# Autodesk Inventor assembly: motor_GM1806-80T_skyProRO
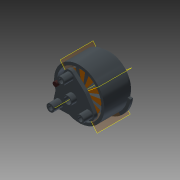
[picture p0: Inventor's stored thumbnail of the model, 180x180]
Saved by Autodesk Inventor 2015 SP1 (Build 190203100, 203)
## iProperties
Created: 2015-08-06
Part Number: motor_GM1806-80T_skyProRO
Document SubType Name: Assembly
Designer: Alexandre Cherpillod
Mass: 18 g
Surface Area: 55.0116 cm^2
Volume: 3.08775 cm^3
Author: Alexandre Cherpillod
## Documents named in this file (3)
- D:\_windows\_github_doc\MAVRIC\Mechanics\myCopter_CAD\Inventor\Gimbal_Brushless\motor_GM1806-80T_skyPro.iam
- D:\_windows\_github_doc\MAVRIC\Mechanics\myCopter_CAD\Inventor\Gimbal_Brushless\motor_GM1806-80T_Skypro_stator.ipt
- D:\_windows\_github_doc\MAVRIC\Mechanics\myCopter_CAD\Inventor\Gimbal_Brushless\motor_GM1806-80T_Skypro_rotor.ipt
## Components (2 placed, 2 different names)
1. motor_GM1806-80T_Skypro_stator:1 — Mate:1, Mate:2
2. motor_GM1806-80T_Skypro_rotor:1 — Mate:1, Mate:2
## Relationships (2: Mate 2)
- Mate:1: motor_GM1806-80T_Skypro_stator:1 ↔ motor_GM1806-80T_Skypro_rotor:1
- Mate:2 (-16.8 mm): motor_GM1806-80T_Skypro_stator:1 ↔ motor_GM1806-80T_Skypro_rotor:1
